# Autodesk Inventor assembly: outer_mirrored
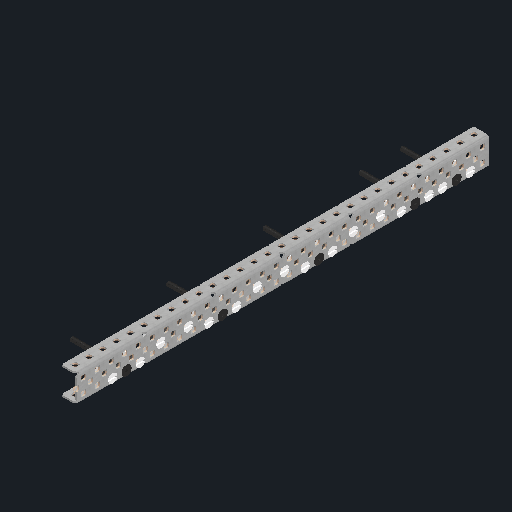
[picture p0: Inventor's stored thumbnail of the model, 512x512]
Saved by Autodesk Inventor 2025 (Build 290162000, 162)
## iProperties
Created: 2024-10-10
Part Number: outer_mirrored
Document SubType Name: Assembly
Designer: Averey Ku
Author: Averey Ku
## Documents named in this file (4)
- D:\vex_robotics_high_stakes\hardware\cad\bots\high_stakes_v2\chassis_v2\drivebay_mirrored\outer_mirrored.iam
- D:\vex_robotics_high_stakes\hardware\cad\bots\high_stakes_v2\chassis_v2\drivebay_mirrored\Alu C 1x2x1x30_mirrored.ipt
- D:\vex_robotics_high_stakes\hardware\cad\bots\high_stakes_v2\chassis_v2\drivebay_mirrored\bearing_flat_w_hardware_mirrored.iam
- D:\vex_robotics_high_stakes\hardware\cad\bots\high_stakes_v2\chassis_v2\drivebay_mirrored\ASScrew Hex Threaded 2.000_mirrored.ipt
## Components (14 placed, 3 different names)
1. Alu C 1x2x1x30_mirrored:1 — Mate:6, Insert:6, Mate:7, Insert:7, Insert:8, Insert:10, Mate:8, Insert:11
2. ASScrew Hex Threaded 2.000_mirrored:1 — Insert:10
3. bearing_flat_w_hardware_mirrored:2 [sub-assembly] — Mate:6, Insert:6
4. ASScrew Hex Threaded 2.000_mirrored:3
5. bearing_flat_w_hardware_mirrored:4 [sub-assembly]
6. ASScrew Hex Threaded 2.000_mirrored:4
7. bearing_flat_w_hardware_mirrored:5 [sub-assembly]
8. bearing_flat_w_hardware_mirrored:1 [sub-assembly] — Mate:7, Insert:7
9. bearing_flat_w_hardware_mirrored:6 [sub-assembly]
10. bearing_flat_w_hardware_mirrored:7 [sub-assembly]
11. bearing_flat_w_hardware_mirrored:3 [sub-assembly] — Mate:8, Insert:11
12. ASScrew Hex Threaded 2.000_mirrored:2 — Insert:8
13. bearing_flat_w_hardware_mirrored:8 [sub-assembly]
14. ASScrew Hex Threaded 2.000_mirrored:5
## Component patterns: (3 elements, first: ASScrew Hex Threaded 2.000_mirrored:1 + bearing_flat_w_hardware_mirrored:2), (3 elements, first: bearing_flat_w_hardware_mirrored:1), (2 elements, first: bearing_flat_w_hardware_mirrored:3 + ASScrew Hex Threaded 2.000_mirrored:2)
## Relationships (8: Insert 5, Mate 3)
- Mate:6: Alu C 1x2x1x30_mirrored:1 ↔ bearing_flat_w_hardware_mirrored:2
- Insert:6: Alu C 1x2x1x30_mirrored:1 ↔ bearing_flat_w_hardware_mirrored:2
- Mate:7: Alu C 1x2x1x30_mirrored:1 ↔ bearing_flat_w_hardware_mirrored:1
- Insert:7: Alu C 1x2x1x30_mirrored:1 ↔ bearing_flat_w_hardware_mirrored:1
- Insert:8 (-1.5875 mm): Alu C 1x2x1x30_mirrored:1 ↔ ASScrew Hex Threaded 2.000_mirrored:2
- Insert:10 (-1.5875 mm): Alu C 1x2x1x30_mirrored:1 ↔ ASScrew Hex Threaded 2.000_mirrored:1
- Mate:8: Alu C 1x2x1x30_mirrored:1 ↔ bearing_flat_w_hardware_mirrored:3
- Insert:11: Alu C 1x2x1x30_mirrored:1 ↔ bearing_flat_w_hardware_mirrored:3
